# Autodesk Inventor assembly: Composit Material Table
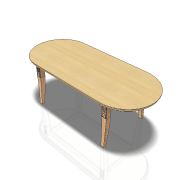
[picture p0: Inventor's stored thumbnail of the model, 180x180]
Saved by Autodesk Inventor 2024 (Build 280153000, 153)
## iProperties
Created: 2020-04-16
Part Number: Composit Material Table
Document SubType Name: Assembly
Designer: SauliusD
Author: SauliusD
## Documents named in this file (11)
- C:\W4INV 2024 Design\PROJECTS\Samples\Composite Material Table\Composite Material Table.iam
- C:\W4INV 2024 Design\PROJECTS\Samples\Composite Material Table\3 Technological Stage Table\Third Technological Stage Table Top Final Processing.ipt
- C:\W4INV 2024 Design\PROJECTS\Samples\Composite Material Table\Leg\Final Leg.ipt
- C:\W4INV 2024 Design\PROJECTS\Samples\Composite Material Table\Cross Frame.ipt
- C:\W4INV 2024 Design\PROJECTS\Samples\Composite Material Table\Along Frame.ipt
- C:\W4INV 2024 Design\PROJECTS\Samples\Composite Material Table\Dowel.ipt
- C:\W4INV 2024 Design\_LIBRARY\Fixed joints\Dowel\DOWEL V2\Dowel 8x30 PB T=19.ipt
- C:\W4INV 2024 Design\PROJECTS\Samples\Composite Material Table\Leg\Front Front Final Leg.ipt
- C:\W4INV 2024 Design\PROJECTS\Samples\Composite Material Table\Leg\Back Left Final Leg_MIR.ipt
- C:\W4INV 2024 Design\PROJECTS\Samples\Composite Material Table\Leg\Front Left  Final Leg_MIR.ipt
- C:\W4INV 2022 Design\LIBRARY\Fixed joints\Dowel\DOWEL V2.ipt
## Components (30 placed, 9 different names)
1. Third Technological Stage Table Top Final Processing:1 — Flush:4, Flush:5, Flush:6, Table bottom:1, Table bottom:2, Table bottom:3, Table bottom:4
2. Final Leg:1 — Flush:1, Flush:2, Flush:3, Flush:7, Flush:8, Flush:9, Nestled Board Plane:9, Nestled Board Plane:11, Nestled Board Plane:13, Nestled Board Plane:15, 2 Axis Plane:1, 2 Axis Plane:2
3. Cross Frame:1 — Pillar Board Plane:9, Pillar Board Plane:10, Pillar Board Plane:13, Pillar Board Plane:14
4. Along Frame:1 — Axis Plane:1, Axis Plane:2, Axis Plane:3, Pillar Board Plane:3, Axis Plane:4, Pillar Board Plane:4, Axis Plane:5, Axis Plane:6, Axis Plane:7, Pillar Board Plane:7, Axis Plane:8, Pillar Board Plane:8, Axis Plane:9, Axis Plane:10, Axis Plane:11, Axis Plane:12, Axis Plane:13, Axis Plane:14, Axis Plane:15, Axis Plane:16
5. Along Frame:2 — Pillar Board Plane:1, Pillar Board Plane:2, Pillar Board Plane:5, Pillar Board Plane:6
6. Cross Frame:2 — Pillar Board Plane:11, Pillar Board Plane:12, Pillar Board Plane:15, Pillar Board Plane:16
7. Final Leg:3 — Flush:12, Flush:13, Flush:14, Flush:15, Flush:16, Flush:17, 1 Axis Plane:1, 1 Axis Plane:3
8. Front Front Final Leg:1 — Flush:29, Mate:66, Mate:67, Flush:30, Mate:68, Mate:69, Nestled Board Plane:1, Nestled Board Plane:3, Nestled Board Plane:5, Nestled Board Plane:7, Nestled Board Plane:10, Nestled Board Plane:12, Nestled Board Plane:14, Nestled Board Plane:16, 2 Axis Plane:3, 2 Axis Plane:4
9. Back Left Final Leg_MIR:1 — Mate:70, Flush:31, Mate:71, Mate:72, Flush:32, Mate:73, 1 Axis Plane:2, 1 Axis Plane:4
10. Front Left  Final Leg_MIR:1 — Flush:33, Mate:74, Flush:34, Flush:35, Mate:75, Flush:36, Nestled Board Plane:2, Nestled Board Plane:4, Nestled Board Plane:6, Nestled Board Plane:8
11. Dowel 8x30 PB T=19:2 — Axis Plane:1, Pillar Board Plane:1, Nestled Board Plane:1
12. Dowel 8x30 PB T=19:3 — Axis Plane:2, Pillar Board Plane:2, Nestled Board Plane:2
13. Dowel 8x30 PB T=19:4 — Axis Plane:3, Pillar Board Plane:3, Nestled Board Plane:3
14. Dowel 8x30 PB T=19:5 — Axis Plane:4, Pillar Board Plane:4, Nestled Board Plane:4
15. Dowel 8x30 PB T=19:6 — Axis Plane:5, Pillar Board Plane:5, Nestled Board Plane:5
16. Dowel 8x30 PB T=19:7 — Axis Plane:6, Pillar Board Plane:6, Nestled Board Plane:6
17. Dowel 8x30 PB T=19:8 — Axis Plane:7, Pillar Board Plane:7, Nestled Board Plane:7
18. Dowel 8x30 PB T=19:9 — Axis Plane:8, Pillar Board Plane:8, Nestled Board Plane:8
19. Dowel 8x30 PB T=19:10 — Axis Plane:9, Pillar Board Plane:9, Nestled Board Plane:9
20. Dowel 8x30 PB T=19:11 — Axis Plane:10, Pillar Board Plane:10, Nestled Board Plane:10
21. Dowel 8x30 PB T=19:12 — Axis Plane:11, Pillar Board Plane:11, Nestled Board Plane:11
22. Dowel 8x30 PB T=19:13 — Axis Plane:12, Pillar Board Plane:12, Nestled Board Plane:12
23. Dowel 8x30 PB T=19:14 — Axis Plane:13, Pillar Board Plane:13, Nestled Board Plane:13
24. Dowel 8x30 PB T=19:15 — Axis Plane:14, Pillar Board Plane:14, Nestled Board Plane:14
25. Dowel 8x30 PB T=19:16 — Axis Plane:15, Pillar Board Plane:15, Nestled Board Plane:15
26. Dowel 8x30 PB T=19:17 — Axis Plane:16, Pillar Board Plane:16, Nestled Board Plane:16
27. Dowel:6 — 2 Axis Plane:1, 1 Axis Plane:1, Table bottom:1
28. Dowel:7 — 2 Axis Plane:2, 1 Axis Plane:2, Table bottom:2
29. Dowel:8 — 2 Axis Plane:3, 1 Axis Plane:3, Table bottom:3
30. Dowel:9 — 2 Axis Plane:4, 1 Axis Plane:4, Table bottom:4
## Relationships (93: Mate 66, Flush 27)
- Flush:1: Final Leg:1
- Flush:2: Final Leg:1
- Flush:3: Final Leg:1
- Flush:4: Third Technological Stage Table Top Final Processing:1
- Flush:5: Third Technological Stage Table Top Final Processing:1
- Flush:6: Third Technological Stage Table Top Final Processing:1
- Flush:7: Final Leg:1
- Flush:8: Final Leg:1
- Flush:9: Final Leg:1
- Flush:12: Final Leg:3
- Flush:13: Final Leg:3
- Flush:14: Final Leg:3
- Flush:15: Final Leg:3
- Flush:16: Final Leg:3
- Flush:17: Final Leg:3
- Flush:29: Front Front Final Leg:1
- Mate:66: Front Front Final Leg:1
- Mate:67: Front Front Final Leg:1
- Flush:30: Front Front Final Leg:1
- Mate:68: Front Front Final Leg:1
- Mate:69: Front Front Final Leg:1
- Mate:70: Back Left Final Leg_MIR:1
- Flush:31: Back Left Final Leg_MIR:1
- Mate:71: Back Left Final Leg_MIR:1
- Mate:72: Back Left Final Leg_MIR:1
- Flush:32: Back Left Final Leg_MIR:1
- Mate:73: Back Left Final Leg_MIR:1
- Flush:33: Front Left  Final Leg_MIR:1
- Mate:74: Front Left  Final Leg_MIR:1
- Flush:34: Front Left  Final Leg_MIR:1
- Flush:35: Front Left  Final Leg_MIR:1
- Mate:75: Front Left  Final Leg_MIR:1
- Flush:36: Front Left  Final Leg_MIR:1
- Axis Plane:1 [Mate]: Along Frame:1 ↔ Dowel 8x30 PB T=19:2
- Pillar Board Plane:1 [Mate] (-9.5 mm): Along Frame:2 ↔ Dowel 8x30 PB T=19:2
- Nestled Board Plane:1 [Mate]: Front Front Final Leg:1 ↔ Dowel 8x30 PB T=19:2
- Axis Plane:2 [Mate]: Along Frame:1 ↔ Dowel 8x30 PB T=19:3
- Pillar Board Plane:2 [Mate] (-9.5 mm): Along Frame:2 ↔ Dowel 8x30 PB T=19:3
- Nestled Board Plane:2 [Mate]: Front Left  Final Leg_MIR:1 ↔ Dowel 8x30 PB T=19:3
- Axis Plane:3 [Mate]: Along Frame:1 ↔ Dowel 8x30 PB T=19:4
- Pillar Board Plane:3 [Mate] (-9.5 mm): Along Frame:1 ↔ Dowel 8x30 PB T=19:4
- Nestled Board Plane:3 [Mate]: Front Front Final Leg:1 ↔ Dowel 8x30 PB T=19:4
- Axis Plane:4 [Mate]: Along Frame:1 ↔ Dowel 8x30 PB T=19:5
- Pillar Board Plane:4 [Mate] (-9.5 mm): Along Frame:1 ↔ Dowel 8x30 PB T=19:5
- Nestled Board Plane:4 [Mate]: Front Left  Final Leg_MIR:1 ↔ Dowel 8x30 PB T=19:5
- Axis Plane:5 [Mate]: Along Frame:1 ↔ Dowel 8x30 PB T=19:6
- Pillar Board Plane:5 [Mate] (-9.5 mm): Along Frame:2 ↔ Dowel 8x30 PB T=19:6
- Nestled Board Plane:5 [Mate]: Front Front Final Leg:1 ↔ Dowel 8x30 PB T=19:6
- Axis Plane:6 [Mate]: Along Frame:1 ↔ Dowel 8x30 PB T=19:7
- Pillar Board Plane:6 [Mate] (-9.5 mm): Along Frame:2 ↔ Dowel 8x30 PB T=19:7
- Nestled Board Plane:6 [Mate]: Front Left  Final Leg_MIR:1 ↔ Dowel 8x30 PB T=19:7
- Axis Plane:7 [Mate]: Along Frame:1 ↔ Dowel 8x30 PB T=19:8
- Pillar Board Plane:7 [Mate] (-9.5 mm): Along Frame:1 ↔ Dowel 8x30 PB T=19:8
- Nestled Board Plane:7 [Mate]: Front Front Final Leg:1 ↔ Dowel 8x30 PB T=19:8
- Axis Plane:8 [Mate]: Along Frame:1 ↔ Dowel 8x30 PB T=19:9
- Pillar Board Plane:8 [Mate] (-9.5 mm): Along Frame:1 ↔ Dowel 8x30 PB T=19:9
- Nestled Board Plane:8 [Mate]: Front Left  Final Leg_MIR:1 ↔ Dowel 8x30 PB T=19:9
- Axis Plane:9 [Mate]: Along Frame:1 ↔ Dowel 8x30 PB T=19:10
- Pillar Board Plane:9 [Mate] (-9.5 mm): Cross Frame:1 ↔ Dowel 8x30 PB T=19:10
- Nestled Board Plane:9 [Mate]: Final Leg:1 ↔ Dowel 8x30 PB T=19:10
- Axis Plane:10 [Mate]: Along Frame:1 ↔ Dowel 8x30 PB T=19:11
- Pillar Board Plane:10 [Mate] (-9.5 mm): Cross Frame:1 ↔ Dowel 8x30 PB T=19:11
- Nestled Board Plane:10 [Mate]: Front Front Final Leg:1 ↔ Dowel 8x30 PB T=19:11
- Axis Plane:11 [Mate]: Along Frame:1 ↔ Dowel 8x30 PB T=19:12
- Pillar Board Plane:11 [Mate] (-9.5 mm): Cross Frame:2 ↔ Dowel 8x30 PB T=19:12
- Nestled Board Plane:11 [Mate]: Final Leg:1 ↔ Dowel 8x30 PB T=19:12
- Axis Plane:12 [Mate]: Along Frame:1 ↔ Dowel 8x30 PB T=19:13
- Pillar Board Plane:12 [Mate] (-9.5 mm): Cross Frame:2 ↔ Dowel 8x30 PB T=19:13
- Nestled Board Plane:12 [Mate]: Front Front Final Leg:1 ↔ Dowel 8x30 PB T=19:13
- Axis Plane:13 [Mate]: Along Frame:1 ↔ Dowel 8x30 PB T=19:14
- Pillar Board Plane:13 [Mate] (-9.5 mm): Cross Frame:1 ↔ Dowel 8x30 PB T=19:14
- Nestled Board Plane:13 [Mate]: Final Leg:1 ↔ Dowel 8x30 PB T=19:14
- Axis Plane:14 [Mate]: Along Frame:1 ↔ Dowel 8x30 PB T=19:15
- Pillar Board Plane:14 [Mate] (-9.5 mm): Cross Frame:1 ↔ Dowel 8x30 PB T=19:15
- Nestled Board Plane:14 [Mate]: Front Front Final Leg:1 ↔ Dowel 8x30 PB T=19:15
- Axis Plane:15 [Mate]: Along Frame:1 ↔ Dowel 8x30 PB T=19:16
- Pillar Board Plane:15 [Mate] (-9.5 mm): Cross Frame:2 ↔ Dowel 8x30 PB T=19:16
- Nestled Board Plane:15 [Mate]: Final Leg:1 ↔ Dowel 8x30 PB T=19:16
- Axis Plane:16 [Mate]: Along Frame:1 ↔ Dowel 8x30 PB T=19:17
- Pillar Board Plane:16 [Mate] (-9.5 mm): Cross Frame:2 ↔ Dowel 8x30 PB T=19:17
- Nestled Board Plane:16 [Mate]: Front Front Final Leg:1 ↔ Dowel 8x30 PB T=19:17
- 2 Axis Plane:1 [Mate]: Final Leg:1 ↔ Dowel:6
- 1 Axis Plane:1 [Mate]: Final Leg:3 ↔ Dowel:6
- Table bottom:1 [Flush]: Third Technological Stage Table Top Final Processing:1 ↔ Dowel:6
- 2 Axis Plane:2 [Mate]: Final Leg:1 ↔ Dowel:7
- 1 Axis Plane:2 [Mate]: Back Left Final Leg_MIR:1 ↔ Dowel:7
- Table bottom:2 [Flush]: Third Technological Stage Table Top Final Processing:1 ↔ Dowel:7
- 2 Axis Plane:3 [Mate]: Front Front Final Leg:1 ↔ Dowel:8
- 1 Axis Plane:3 [Mate]: Final Leg:3 ↔ Dowel:8
- Table bottom:3 [Flush]: Third Technological Stage Table Top Final Processing:1 ↔ Dowel:8
- 2 Axis Plane:4 [Mate]: Front Front Final Leg:1 ↔ Dowel:9
- 1 Axis Plane:4 [Mate]: Back Left Final Leg_MIR:1 ↔ Dowel:9
- Table bottom:4 [Flush]: Third Technological Stage Table Top Final Processing:1 ↔ Dowel:9
